# Autodesk Inventor assembly: ChainInterLink-ver1-1111-2018
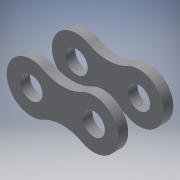
[picture p0: Inventor's stored thumbnail of the model, 180x180]
Saved by Autodesk Inventor 2017 (Build 210142000, 142)
## iProperties
Created: 2018-01-27
Part Number: ChainInterLink-ver1-1111-2018
Document SubType Name: Assembly
Designer: 764368
Author: 764368
## Documents named in this file (2)
- E:\GrabCAD\Power Hawks CAD\VEXpro Resources\Versa Motion\Chain\ChainInterLink-ver1-1111-2018.iam
- E:\GrabCAD\Power Hawks CAD\VEXpro Resources\Versa Motion\Chain\Chain Link.ipt
## Components (2 placed, 1 different names)
1. Chain Link:1 — Mate:1, Mate:2, Mate:3
2. Chain Link:2 — Mate:1, Mate:2, Mate:3
## Relationships (3: Mate 3)
- Mate:1 (3.6068 mm): Chain Link:1 ↔ Chain Link:2
- Mate:2: Chain Link:1 ↔ Chain Link:2
- Mate:3: Chain Link:1 ↔ Chain Link:2
